# Autodesk Inventor assembly: gimbal_v2
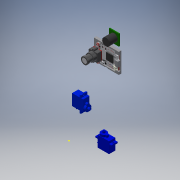
[picture p0: Inventor's stored thumbnail of the model, 180x180]
Saved by Autodesk Inventor 2019 (Build 230136000, 136)
## iProperties
Created: 2020-03-15
Part Number: gimbal_v2
Document SubType Name: Assembly
Designer: Pulag
Author: Pulag
## Documents named in this file (7)
- C:\Users\Pulag\Documents\GitHub\24th_TDK_Project_D5\CAD\frame\gimbal_v2.iam
- C:\Users\Pulag\Documents\GitHub\24th_TDK_Project_D5\CAD\Syno_borad_3D\匯出\SG90.ipt
- C:\Users\Pulag\Documents\GitHub\24th_TDK_Project_D5\CAD\frame\frame3.ipt
- C:\Users\Pulag\Documents\GitHub\24th_TDK_Project_D5\CAD\frame\frame4.ipt
- C:\Users\Pulag\Documents\GitHub\24th_TDK_Project_D5\CAD\CAD file\OpenMV H7\openmv4_h7.iam
- C:\Users\Pulag\Documents\GitHub\24th_TDK_Project_D5\CAD\frame\SONIC.ipt
- C:\Users\Pulag\Documents\GitHub\24th_TDK_Project_D5\CAD\frame\part1.ipt
## Components (7 placed, 6 different names)
1. SG90:1 — Flush:1, Flush:2, Flush:3
2. SG90:2 — Mate:10, Flush:2
3. frame3:1
4. frame4:1
5. openmv4_h7:1 [sub-assembly] — Flush:1, Mate:11, Mate:12, Mate:13
6. SONIC:1 — Flush:3
7. part1:1 — Mate:11, Mate:12, Mate:13
## Relationships (7: Mate 4, Flush 3)
- Mate:10: SG90:2
- Flush:1: SG90:1 ↔ openmv4_h7:1
- Flush:2: SG90:1 ↔ SG90:2
- Flush:3: SG90:1 ↔ SONIC:1
- Mate:11: openmv4_h7:1 ↔ part1:1
- Mate:12: openmv4_h7:1 ↔ part1:1
- Mate:13: openmv4_h7:1 ↔ part1:1
